# Autodesk Inventor assembly: ASM_guia_eliptica
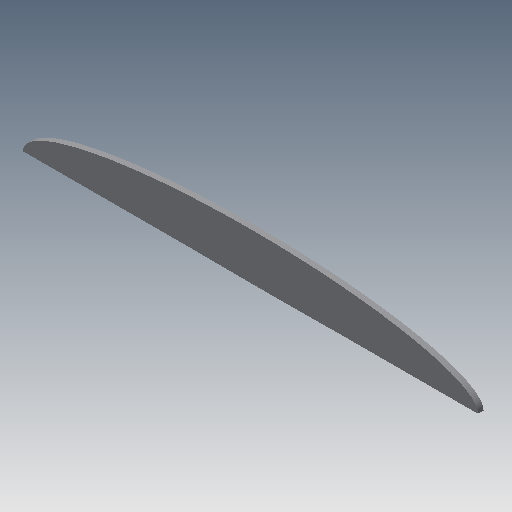
[picture p0: Inventor's stored thumbnail of the model, 512x512]
Saved by Autodesk Inventor 2019 (Build 230136000, 136)
## iProperties
Created: 2019-11-05
Part Number: ASM_guia_eliptica
Document SubType Name: Assembly
Designer: Charlie
Author: Charlie
## Documents named in this file (3)
- C:\Users\user\OneDrive\Carlos_2\02 TRABAJOS\MULTIPLO\Conveyor\Torno_rodillos\ASM_guia_eliptica.iam
- C:\Users\user\OneDrive\Carlos_2\02 TRABAJOS\MULTIPLO\Conveyor\Torno_rodillos\Apoyo guia eliptica.ipt
- C:\Users\user\OneDrive\Carlos_2\02 TRABAJOS\MULTIPLO\Conveyor\Torno_rodillos\Guia eliptica_1.ipt
## Components (2 placed, 2 different names)
1. Apoyo guia eliptica:1
2. Guia eliptica_1:1
## Relationships (2: RevoluteJoint 1, Mate 1)
- [RevoluteJoint]: Apoyo guia eliptica:1 ↔ Guia eliptica_1:1
- [Mate]: Apoyo guia eliptica:1 ↔ Guia eliptica_1:1
